# Autodesk Inventor assembly: Assy_upper_arm
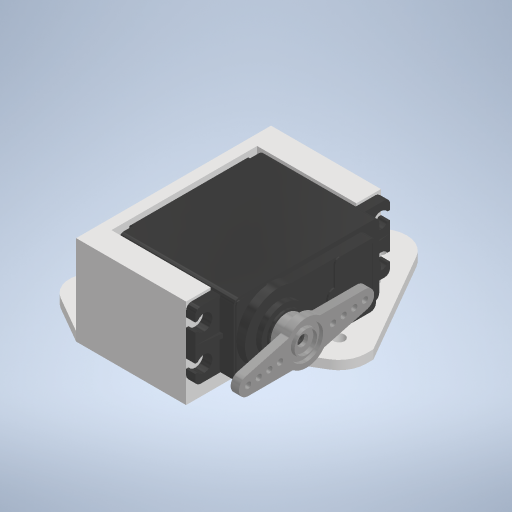
[picture p0: Inventor's stored thumbnail of the model, 512x512]
Saved by Autodesk Inventor 2024.1 (Build 281209000, 209)
## iProperties
Created: 2025-03-03
Part Number: Assy_upper_arm
Document SubType Name: Assembly
Designer: hibik
Author: hibik
## Documents named in this file (5)
- C:\Users\hibik\Documents\Robomech\RESCUE\ORCA\hard\arm\Assy_upper_arm.iam
- C:\Users\hibik\Documents\Robomech\RESCUE\ORCA\hard\arm\upper_arm_base.ipt
- C:\Users\hibik\Documents\Robomech\RESCUE\ORCA\hard\std_parts\FS5103B.ipt
- C:\Users\hibik\Documents\Robomech\RESCUE\ORCA\hard\std_parts\feetech_servohone.ipt
- C:\Users\hibik\Documents\Robomech\RESCUE\ORCA\hard\std_parts\bearing_6_10_3.ipt
## Components (4 placed, 4 different names)
1. upper_arm_base:1 — メイト:1, メイト:2, メイト:3, 挿入:2
2. FS5103B:1 — メイト:1, メイト:2, メイト:3, 挿入:1
3. feetech_servohone:1 — 挿入:1
4. bearing_6_10_3:1 — 挿入:2
## Relationships (5: Mate 3, Insert 2)
- メイト:1 [Mate]: upper_arm_base:1 ↔ FS5103B:1
- メイト:2 [Mate]: upper_arm_base:1 ↔ FS5103B:1
- メイト:3 [Mate]: upper_arm_base:1 ↔ FS5103B:1
- 挿入:1 [Insert]: FS5103B:1 ↔ feetech_servohone:1
- 挿入:2 [Insert]: upper_arm_base:1 ↔ bearing_6_10_3:1
